# Autodesk Inventor assembly: 100ml Bottle and Lid
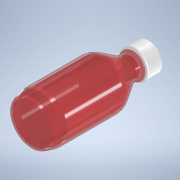
[picture p0: Inventor's stored thumbnail of the model, 180x180]
Saved by Autodesk Inventor 2021 (Build 250183000, 183)
## iProperties
Created: 2020-04-02
Part Number: 100ml Bottle and Lid
Document SubType Name: Assembly
Designer: jgray
Author: jgray
## Documents named in this file (3)
- M:\Printed Electronics\Gas Sensors\Prototypes\Prototype II -Cartridge Reader V2\100ml Bottle and Lid.iam
- M:\Printed Electronics\Gas Sensors\Prototypes\Prototype II -Cartridge Reader V2\100ml Bottle 2 lid.ipt
- M:\Printed Electronics\Gas Sensors\Prototypes\Prototype II -Cartridge Reader V2\100ml Bottle 2.ipt
## Components (2 placed, 2 different names)
1. 100ml Bottle 2 lid:1 — Mate:1, Mate:2
2. 100ml Bottle 2:1 — Mate:1, Mate:2
## Relationships (2: Mate 2)
- Mate:1: 100ml Bottle 2 lid:1 ↔ 100ml Bottle 2:1
- Mate:2: 100ml Bottle 2 lid:1 ↔ 100ml Bottle 2:1
